# Autodesk Inventor assembly: Assembly1
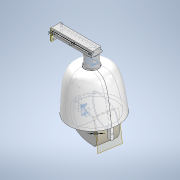
[picture p0: Inventor's stored thumbnail of the model, 180x180]
Saved by Autodesk Inventor 2021.1 (Build 251245010, 245A)
## iProperties
Created: 2023-07-02
Part Number: Assembly1
Document SubType Name: Assembly
Designer: Drake
Author: Drake
## Documents named in this file (5)
- C:\bkp\FYPDESIGN\Assembly1.iam
- C:\bkp\FYPDESIGN\TopBracket.ipt
- C:\bkp\FYPDESIGN\Motor.ipt
- C:\bkp\FYPDESIGN\EnclosingRevolver.ipt
- C:\bkp\FYPDESIGN\CameraHolder2.ipt
## Components (5 placed, 4 different names)
1. TopBracket:1 — Mate:1, Mate:2, Mate:4
2. Motor:3 — Mate:1, Mate:2, Rotational:1
3. EnclosingRevolver:1 — Rotational:1, Mate:3, Rotational:2, Mate:4
4. CameraHolder2:1 — Mate:3
5. Motor:4 — Rotational:2
## Relationships (6: Mate 4, RevoluteJoint 2)
- Mate:1: TopBracket:1 ↔ Motor:3
- Mate:2: TopBracket:1 ↔ Motor:3
- Rotational:1 [RevoluteJoint] (-2.54 mm): Motor:3 ↔ EnclosingRevolver:1
- Mate:3: EnclosingRevolver:1 ↔ CameraHolder2:1
- Rotational:2 [RevoluteJoint]: EnclosingRevolver:1 ↔ Motor:4
- Mate:4: TopBracket:1 ↔ EnclosingRevolver:1
